# Autodesk Inventor assembly: Сборка_опт_зонд_с_датчиком
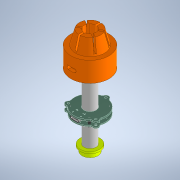
[picture p0: Inventor's stored thumbnail of the model, 180x180]
Saved by Autodesk Inventor 2021 (Build 250183000, 183)
## iProperties
Created: 2024-03-30
Part Number: Сборка_опт_зонд_с_датчиком
Document SubType Name: Assembly
Designer: Мария
Author: Мария
## Documents named in this file (6)
- D:\Documents\Inventor\Разводка печатных плат\Сборка_опт_зонд_с_датчиком.iam
- D:\Documents\Inventor\Разводка печатных плат\Оптический датчик.ipt
- D:\Documents\Inventor\Разводка печатных плат\Упор.ipt
- D:\Documents\Inventor\Разводка печатных плат\Цанга_держатель.ipt
- D:\Documents\Inventor\Разводка печатных плат\PCB\pressure_sensor_sensor2.iam
- D:\Documents\Inventor\Разводка печатных плат\PCB\pressure_sensor_logic2_.iam
## Components (5 placed, 5 different names)
1. Оптический датчик:1 — Совмещение:6, Совмещение:11, Совмещение:12, Совмещение:18, Совмещение:19, Совмещение:20, Совмещение:23
2. Упор:1 — Совмещение:12, Совмещение:18
3. Цанга_держатель:1 — Совмещение:6, Совмещение:11
4. pressure_sensor_sensor2:1 [sub-assembly] — Совмещение:19, Совмещение:21, Совмещение:22
5. pressure_sensor_logic2_:1 [sub-assembly] — Совмещение:20, Совмещение:21, Совмещение:22, Совмещение:23
## Relationships (9: Mate 9)
- Совмещение:6 [Mate]: Оптический датчик:1 ↔ Цанга_держатель:1
- Совмещение:11 [Mate]: Оптический датчик:1 ↔ Цанга_держатель:1
- Совмещение:12 [Mate]: Оптический датчик:1 ↔ Упор:1
- Совмещение:18 [Mate]: Оптический датчик:1 ↔ Упор:1
- Совмещение:19 [Mate]: Оптический датчик:1 ↔ pressure_sensor_sensor2:1
- Совмещение:20 [Mate]: Оптический датчик:1 ↔ pressure_sensor_logic2_:1
- Совмещение:21 [Mate]: pressure_sensor_sensor2:1 ↔ pressure_sensor_logic2_:1
- Совмещение:22 [Mate] (4 mm): pressure_sensor_sensor2:1 ↔ pressure_sensor_logic2_:1
- Совмещение:23 [Mate]: Оптический датчик:1 ↔ pressure_sensor_logic2_:1
